# Autodesk Inventor assembly: Lego Maniam
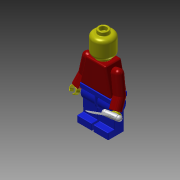
[picture p0: Inventor's stored thumbnail of the model, 180x180]
Saved by Autodesk Inventor 2013 (Build 170138000, 138)
## iProperties
Created: 2013-09-07
Part Number: Lego Maniam
Document SubType Name: Assembly
Designer: 200395375
Author: 200395375
## Documents named in this file (10)
- C:\Users\200395375\Desktop\Favourites\AutoDesk Projects\1. Inventor\2.Assembly\2. LegoMan\Lego Man with sword.iam
- C:\Users\200395375\Desktop\Favourites\AutoDesk Projects\1. Inventor\2.Assembly\2. LegoMan\Components\Lego Joint.ipt
- C:\Users\200395375\Desktop\Favourites\AutoDesk Projects\1. Inventor\2.Assembly\2. LegoMan\Components\Lego Body.ipt
- C:\Users\200395375\Desktop\Favourites\AutoDesk Projects\1. Inventor\2.Assembly\2. LegoMan\Components\Lego Hand.ipt
- C:\Users\200395375\Desktop\Favourites\AutoDesk Projects\1. Inventor\2.Assembly\2. LegoMan\Components\Lego Head.ipt
- C:\Users\200395375\Desktop\Favourites\AutoDesk Projects\1. Inventor\2.Assembly\2. LegoMan\Components\Lego Leg(left).ipt
- C:\Users\200395375\Desktop\Favourites\AutoDesk Projects\1. Inventor\2.Assembly\2. LegoMan\Components\Lego Leg(Right).ipt
- C:\Users\200395375\Desktop\Favourites\AutoDesk Projects\1. Inventor\2.Assembly\2. LegoMan\Components\Lego Arm(left).ipt
- C:\Users\200395375\Desktop\Favourites\AutoDesk Projects\1. Inventor\2.Assembly\2. LegoMan\Components\Lego Arm(right).ipt
- C:\Users\200395375\Desktop\Favourites\AutoDesk Projects\1. Inventor\2.Assembly\2. LegoMan\Lego Sword.ipt
## Components (10 placed, 9 different names)
1. Lego Joint:1 — Insert:2, Insert:3, Insert:4
2. Lego Body:1 — Insert:1, Insert:4, Insert:5, Insert:6
3. Lego Hand:1 — Insert:8
4. Lego Head:1 — Insert:1
5. Lego Leg(left):1 — Insert:3
6. Lego Leg(Right):1 — Insert:2
7. Lego Hand:2 — Insert:7, Insert:9
8. Lego Arm(left):1 — Insert:5, Insert:8
9. Lego Arm(right):1 — Insert:6, Insert:7
10. Lego Sword:1 — Insert:9
## Relationships (9: Insert 9)
- Insert:1: Lego Body:1 ↔ Lego Head:1
- Insert:2: Lego Joint:1 ↔ Lego Leg(Right):1
- Insert:3: Lego Joint:1 ↔ Lego Leg(left):1
- Insert:4: Lego Joint:1 ↔ Lego Body:1
- Insert:5: Lego Body:1 ↔ Lego Arm(left):1
- Insert:6: Lego Body:1 ↔ Lego Arm(right):1
- Insert:7: Lego Hand:2 ↔ Lego Arm(right):1
- Insert:8: Lego Hand:1 ↔ Lego Arm(left):1
- Insert:9: Lego Hand:2 ↔ Lego Sword:1
